# Autodesk Inventor assembly: V0-UmbilicalBoardRevA
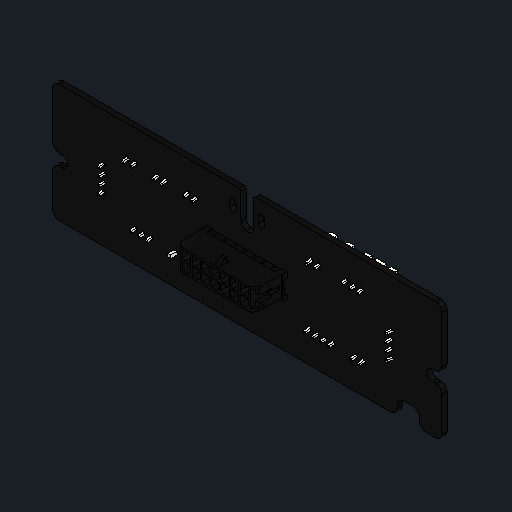
[picture p0: Inventor's stored thumbnail of the model, 512x512]
Saved by Autodesk Inventor 2025.1 (Build 291241020, 241B)
## iProperties
Company: A Company
Created: 2021-04-21
Part Number: V0-UmbilicalBoardRevA
Description: KiCad electronic assembly
Document SubType Name: Assembly
Designer: Joshua Eah
Authority: Unknown
Sending System: KiCad to STEP converter
Preprocessor: Open CASCADE STEP processor 6.9
Title: V0-UmbilicalBoardRevA.step
Author: An Author
## Documents named in this file (7)
- C:\Users\Joshua Eah\Documents\Voron 0.2\CAD\Master Assembly\Frame\Parts\V0-UmbilicalBoardRevA.iam
- C:\Users\Joshua Eah\Documents\Voron 0.2\CAD\Master Assembly\Frame\Parts\COMPOUND.ipt
- C:\Users\Joshua Eah\Documents\Voron 0.2\CAD\Master Assembly\Frame\Parts\SOLID_5.ipt
- C:\Users\Joshua Eah\Documents\Voron 0.2\CAD\Master Assembly\Frame\Parts\SOLID.ipt
- C:\Users\Joshua Eah\Documents\Voron 0.2\CAD\Master Assembly\Frame\Parts\SOLID_4.ipt
- C:\Users\Joshua Eah\Documents\Voron 0.2\CAD\Master Assembly\Frame\Parts\SOLID_2.ipt
- C:\Users\Joshua Eah\Documents\Voron 0.2\CAD\Master Assembly\Frame\Parts\SOLID_3.ipt
## Components (13 placed, 13 different names)
1. 2
2. 8
3. 9
4. 10
5. 12
6. 13
7. 15
8. 17
9. 18
10. 19
11. 20
12. 21
13. 24
## Named parameters: Finish1_Area = 95.2871
note: some values were not read from the file. Shown as the stored number, unit unknown: "Finish1_Area".
